# Autodesk Inventor assembly: 1 Pl Hinge with Wood Screws; Cup with Wood Screws
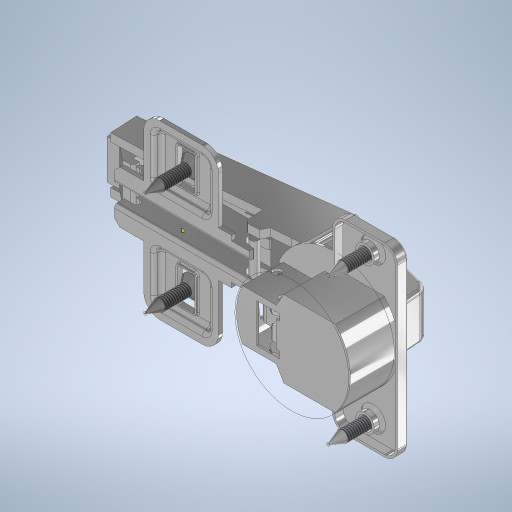
[picture p0: Inventor's stored thumbnail of the model, 512x512]
Saved by Autodesk Inventor 2024 (Build 280153000, 153)
## iProperties
Created: 2014-01-09
Part Number: 1 Pl Hinge with Wood Screws; Cup with Wood Screws
Document SubType Name: Assembly
Designer: G. Kazokaitis
Author: G. Kazokaitis
## Documents named in this file (13)
- C:\W4INV 2024 Design\LIBRARY\Hinges\ONE PLANE HINGE.iam
- C:\W4INV 2024 Design\LIBRARY\Hinges\Parts\One plane hinge\Lever.ipt
- C:\W4INV 2024 Design\LIBRARY\Hinges\Parts\One plane hinge\Linkage.ipt
- C:\W4INV 2024 Design\LIBRARY\Hinges\Parts\One plane hinge\1 Pl Hinge and Plate\1 Pl Hinge and Plate with Wood Screws.ipt
- C:\W4INV 2024 Design\LIBRARY\Hinges\Parts\One plane hinge\1 Pl Hinge and Plate.ipt
- C:\W4INV 2024 Design\LIBRARY\Hinges\Parts\One plane hinge\Cup for 1 Pl Hinge\Cup for 1 Pl hinge with Wood Screws.ipt
- C:\W4INV 2024 Design\LIBRARY\Hinges\Parts\One plane hinge\Cup for 1 Pl Hinge.ipt
- 1 Pl Hinge with Euro Screws(_SC) Cup with Knock-Ins.iam
- 1 Pl Hinge with Euro Screws(_SC) Cup with Wood Screws.iam
- 1 Pl Hinge with Split Dowels(_SC) Cup with Knock-Ins.iam
- 1 Pl Hinge with Split Dowels(_SC) Cup with Wood Screws.iam
- 1 Pl Hinge with Wood Screws(_SC) Cup with Knock-Ins.iam
- 1 Pl Hinge with Wood Screws(_SC) Cup with Wood Screws.iam
## Components (4 placed, 4 different names)
1. 1 Pl Hinge and Plate with Wood Screws:1
2. Lever:1
3. Linkage:1
4. Cup for 1 Pl hinge with Wood Screws:1
## Relationships (11: Mate 7, Flush 3, Angle 1)
- [Flush]: 1 Pl Hinge and Plate with Wood Screws:1
- [Flush]: 1 Pl Hinge and Plate with Wood Screws:1
- [Flush]: 1 Pl Hinge and Plate with Wood Screws:1
- [Mate]: 1 Pl Hinge and Plate with Wood Screws:1 ↔ Lever:1
- [Mate] (0.075 mm): 1 Pl Hinge and Plate with Wood Screws:1 ↔ Lever:1
- [Mate]: 1 Pl Hinge and Plate with Wood Screws:1 ↔ Linkage:1
- [Mate]: 1 Pl Hinge and Plate with Wood Screws:1 ↔ Linkage:1
- [Mate]: Lever:1 ↔ Cup for 1 Pl hinge with Wood Screws:1
- [Mate]: Linkage:1 ↔ Cup for 1 Pl hinge with Wood Screws:1
- [Mate] (1.1 mm): Lever:1 ↔ Cup for 1 Pl hinge with Wood Screws:1
- [Angle] (90 deg): 1 Pl Hinge and Plate with Wood Screws:1 ↔ Cup for 1 Pl hinge with Wood Screws:1
